# Autodesk Inventor assembly: 53
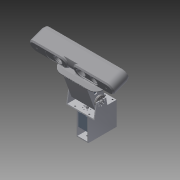
[picture p0: Inventor's stored thumbnail of the model, 180x180]
Saved by Autodesk Inventor 2013 (Build 170138000, 138)
## iProperties
Created: 2014-04-04
Part Number: 53
Document SubType Name: Assembly
Designer: andou
Mass: 334.407 g
Surface Area: 865.333 cm^2
Volume: 252.414 cm^3
Density: 1.32484 g/cm^3
Author: andou
Title: Head
## Documents named in this file (12)
- C:\Users\andou\Documents\Inventor\RoboticsProject\project_4\Robot\Head\Head.iam
- C:\Users\andou\Documents\Inventor\RoboticsProject\project_4\Robot\All Common\Long_Serial_Case.ipt
- C:\Users\andou\Documents\Inventor\RoboticsProject\project_4\Robot\All Common\KRS-2542HV.ipt
- C:\Users\andou\Documents\Inventor\RoboticsProject\project_4\Robot\All Common\Low_Height_Horn.ipt
- C:\Users\andou\Documents\Inventor\RoboticsProject\project_4\Robot\All Common\Bracket.ipt
- C:\Users\andou\Documents\Inventor\RoboticsProject\project_4\Robot\All Common\Serial_Case.ipt
- C:\Users\andou\Documents\Inventor\RoboticsProject\project_4\Robot\All Common\Nylon_Nat(M4).ipt
- C:\Users\andou\Documents\Inventor\RoboticsProject\project_4\Robot\All Common\Washer(M4).ipt
- C:\Users\andou\Documents\Inventor\RoboticsProject\project_4\Robot\All Common\Cap(M4-15).ipt
- C:\Users\andou\Documents\Inventor\RoboticsProject\project_4\Robot\All Common\Cap(M3-6).ipt
- C:\Users\andou\Documents\Inventor\RoboticsProject\project_4\Robot\Free_Horn\Low Free Horn.iam
- C:\Users\andou\Documents\Inventor\RoboticsProject\project_4\Robot\Head\Xtion Pro.ipt
## Components (14 placed, 11 different names)
1. Long_Serial_Case:1 — 挿入:1, 挿入:2, 角度:1
2. KRS-2542HV:1 — 挿入:1, 挿入:2, 挿入:3
3. Low_Height_Horn:1 — 挿入:3, 挿入:7, 挿入:8, 挿入:13
4. Bracket:1 — 挿入:7, 挿入:8, 挿入:15, 挿入:16, 挿入:17
5. Serial_Case:1 — 挿入:5, 挿入:6, 挿入:9, 挿入:12, メイト:1, フラッシュ:1, メイト:2, 角度:1
6. KRS-2542HV:2 — 挿入:4, 挿入:5, 挿入:6
7. Low_Height_Horn:2 — 挿入:4, 挿入:14, 挿入:15, 挿入:17
8. Nylon_Nat(M4):1 — 挿入:11
9. Washer(M4):1 — 挿入:11, 挿入:12
10. Cap(M4-15):1 — 挿入:10
11. Cap(M3-6):1 — 挿入:13
12. Cap(M3-6):2 — 挿入:14
13. Low Free Horn:1 [sub-assembly] — 挿入:9, 挿入:10, 挿入:16
14. Xtion Pro:1 — メイト:1, フラッシュ:1, メイト:2
## Relationships (21: Insert 17, Mate 2, Flush 1, Angle 1)
- 挿入:1 [Insert]: Long_Serial_Case:1 ↔ KRS-2542HV:1
- 挿入:2 [Insert]: Long_Serial_Case:1 ↔ KRS-2542HV:1
- 挿入:3 [Insert]: KRS-2542HV:1 ↔ Low_Height_Horn:1
- 挿入:4 [Insert]: KRS-2542HV:2 ↔ Low_Height_Horn:2
- 挿入:5 [Insert]: Serial_Case:1 ↔ KRS-2542HV:2
- 挿入:6 [Insert]: Serial_Case:1 ↔ KRS-2542HV:2
- 挿入:7 [Insert]: Low_Height_Horn:1 ↔ Bracket:1
- 挿入:8 [Insert]: Low_Height_Horn:1 ↔ Bracket:1
- 挿入:9 [Insert]: Serial_Case:1 ↔ Low Free Horn:1
- 挿入:10 [Insert]: Cap(M4-15):1 ↔ Low Free Horn:1
- 挿入:11 [Insert]: Nylon_Nat(M4):1 ↔ Washer(M4):1
- 挿入:12 [Insert]: Serial_Case:1 ↔ Washer(M4):1
- 挿入:13 [Insert]: Low_Height_Horn:1 ↔ Cap(M3-6):1
- 挿入:14 [Insert]: Low_Height_Horn:2 ↔ Cap(M3-6):2
- 挿入:15 [Insert]: Bracket:1 ↔ Low_Height_Horn:2
- 挿入:16 [Insert]: Bracket:1 ↔ Low Free Horn:1
- 挿入:17 [Insert]: Bracket:1 ↔ Low_Height_Horn:2
- メイト:1 [Mate]: Serial_Case:1 ↔ Xtion Pro:1
- フラッシュ:1 [Flush]: Serial_Case:1 ↔ Xtion Pro:1
- メイト:2 [Mate] (5 mm): Serial_Case:1 ↔ Xtion Pro:1
- 角度:1 [Angle] (340 deg): Long_Serial_Case:1 ↔ Serial_Case:1
